# Autodesk Inventor assembly: Assembly.
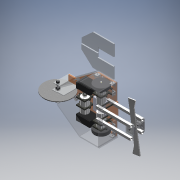
[picture p0: Inventor's stored thumbnail of the model, 180x180]
Saved by Autodesk Inventor 2019 (Build 230136000, 136)
## iProperties
Created: 2018-08-16
Part Number: Assembly.
Document SubType Name: Assembly
Designer: andres2416
Author: andres2416
## Documents named in this file (26)
- C:\Users\garstka1245\Downloads\bot\full-bot-assembly.iam
- C:\Users\garstka1245\Downloads\bot\Electronics\battery.ipt
- C:\Users\garstka1245\Downloads\bot\Motor Mount H\motor-mount-h-E30-bot.ipt
- C:\Users\garstka1245\Downloads\bot\Motor Mount H\motor-mount-h-E30-top.ipt
- C:\Users\garstka1245\Downloads\bot\Mechanicals\motor-E30-400.ipt
- C:\Users\garstka1245\Downloads\bot\Structure\bar-aluminium.ipt
- C:\Users\garstka1245\Downloads\bot\Structure\standoff.ipt
- C:\Users\garstka1245\Downloads\bot\Weapon Saw\wall-side-saw.ipt
- C:\Users\garstka1245\Downloads\bot\Weapon Saw\wall-saw-support.ipt
- C:\Users\garstka1245\Downloads\bot\Weapon Saw\wall-side-saw-hole.ipt
- C:\Users\garstka1245\Downloads\bot\Weapon Saw\weapon-saw.ipt
- C:\Users\garstka1245\Downloads\bot\Mechanicals\wheel-6in.ipt
- C:\Users\garstka1245\Downloads\bot\Weapon Saw\axle-saw.ipt
- C:\Users\garstka1245\Downloads\bot\Shell\base\base.ipt
- C:\Users\garstka1245\Downloads\bot\Shell\second-layer\platform.ipt
- C:\Users\garstka1245\Downloads\bot\Mechanicals\gear-vex.ipt
- C:\Users\garstka1245\Downloads\bot\Weapon Saw\axle-shaft-collar-saw.ipt
- C:\Users\garstka1245\Downloads\bot\Weapon Spinner\mount-point.ipt
- C:\Users\garstka1245\Downloads\bot\Weapon Spinner\axle-spinner.ipt
- C:\Users\garstka1245\Downloads\bot\Weapon Spinner\weapon-spinner.ipt
- C:\Users\garstka1245\Downloads\bot\Shell\wall-parts\wall-spinner.ipt
- C:\Users\garstka1245\Downloads\bot\Shell\wall-parts\wall-side.ipt
- C:\Users\garstka1245\Downloads\bot\Shell\wall-parts\wall-angled.ipt
- C:\Users\garstka1245\Downloads\bot\Structure\bracket-aluminium.ipt
- C:\Users\garstka1245\Downloads\bot\Motor Mount V\motor-mount-v-E30.ipt
- C:\Users\garstka1245\Downloads\bot\Mechanicals\pillowblock.ipt
## Components (61 placed, 25 different names)
1. battery:1 — Mate:116
2. battery:3 — Mate:115
3. wheel-6in:2 — Mate:89, Mate:124
4. wheel-6in:1 — Mate:105, Mate:125
5. gear-vex:1 — Mate:58, Flush:14, Rotation:1, Rotation:2, Rotation:4, Mate:126
6. gear-vex:2 — Mate:92, Flush:14, Rotation:1, Flush:15
7. pillowblock:1 — Mate:112, Mate:113
8. pillowblock:2 — Mate:110, Mate:111, Angle:1
9. motor-E30-400:1 — Mate:101, Mate:102, Mate:105, Flush:18, Mate:125
10. motor-E30-400:2 — Mate:87, Mate:88, Mate:89, Flush:17, Mate:124
11. motor-E30-400:3 — Mate:21, Mate:23, Mate:92, Flush:15, Flush:16
12. motor-mount-h-E30-bot:1 — Mate:96, Mate:97, Mate:98, Mate:99, Mate:102, Mate:107
13. motor-mount-h-E30-bot:2 — Mate:93, Mate:94, Mate:95, Mate:100, Mate:101, Mate:106, Flush:18
14. motor-mount-h-E30-top:2 — Mate:79, Mate:80, Mate:81
15. motor-mount-h-E30-bot:3 — Mate:79, Mate:80, Mate:81, Mate:86, Mate:88, Mate:104
16. motor-mount-h-E30-top:3 — Mate:82, Mate:83, Mate:84
17. motor-mount-h-E30-bot:4 — Mate:82, Mate:83, Mate:84, Mate:85, Mate:87, Mate:103, Flush:17
18. motor-mount-h-E30-bot:5 — Mate:23, Mate:24, Mate:25, Mate:27, Mate:91, Mate:122
19. motor-mount-h-E30-top:7 — Mate:25, Mate:27, Mate:122, Flush:16
20. motor-mount-h-E30-bot:6 — Mate:21, Mate:22, Mate:26, Mate:28, Mate:90, Mate:121
21. motor-mount-h-E30-top:8 — Mate:26, Mate:28, Mate:121
22. motor-mount-h-E30-top:5 — Mate:96, Mate:97, Mate:98
23. motor-mount-h-E30-top:6 — Mate:93, Mate:94, Mate:95
24. motor-mount-v-E30:1 — Mate:118
25. platform:2 — Angle:3, Mate:119
26. platform:1 — Angle:2, Mate:120
27. base:1 — Mate:1, Mate:2, Mate:3, Mate:4, Mate:5, Mate:6, Mate:7, Mate:8, Mate:9, Mate:10, Mate:11, Mate:12, Mate:13, Mate:14, Mate:15, Mate:16, Mate:17, Mate:18, Mate:19, Mate:22, Mate:24, Mate:46, Mate:47, Mate:48, Mate:51, Mate:52, Mate:53, Mate:62, Mate:65, Mate:66, Mate:67, Flush:4, Flush:5, Mate:71, Mate:73, Mate:76, Mate:85, Mate:86, Mate:90, Mate:91, Mate:99, Mate:100, Mate:103, Mate:104, Mate:106, Mate:107, Flush:10, Mate:108, Flush:11, Flush:13, Mate:109, Mate:115, Mate:116, Mate:118, Mate:119, Mate:120
28. wall-side:1 — Mate:73, Mate:74, Mate:75, Angle:3
29. wall-side:2 — Mate:60, Mate:61, Mate:62, Angle:2
30. wall-spinner:1 — Mate:76, Mate:77, Mate:78
31. wall-angled:2 — Mate:70, Mate:71, Mate:72
32. wall-angled:1 — Mate:63, Mate:64, Mate:65
33. standoff:4 — Mate:29, Mate:35, Mate:38, Mate:39
34. standoff:3 — Mate:31, Mate:33
35. standoff:2 — Mate:36, Mate:43
36. standoff:1 — Mate:37, Mate:40, Mate:41, Mate:42
37. bar-aluminium:1 — Mate:33, Mate:35, Mate:38, Flush:6, Flush:7, Mate:68
38. bar-aluminium:2 — Mate:36, Mate:37, Mate:40, Mate:51, Mate:52, Mate:53, Mate:114
39. bar-aluminium:3 — Mate:29, Mate:31, Mate:39, Mate:46, Mate:47, Mate:48, Flush:8, Flush:9
40. bar-aluminium:4 — Mate:41, Mate:42, Mate:43
41. bracket-aluminium:1 — Mate:15, Mate:64, Mate:66
42. bracket-aluminium:2 — Mate:12, Mate:16, Mate:63
43. bracket-aluminium:3 — Mate:11, Mate:14, Mate:72
44. bracket-aluminium:4 — Mate:6, Mate:8, Mate:70
45. bracket-aluminium:5 — Mate:9, Mate:19, Mate:78
46. bracket-aluminium:6 — Mate:1, Mate:2, Mate:77
47. bracket-aluminium:7 — Mate:10, Mate:18, Mate:61
48. bracket-aluminium:8 — Mate:13, Mate:17, Mate:60
49. bracket-aluminium:9 — Mate:3, Mate:4, Mate:74
50. bracket-aluminium:10 — Mate:5, Mate:7, Mate:75
51. wall-side-saw-hole:1 — Mate:55, Flush:10, Mate:108, Flush:11, Flush:12, Mate:126, Mate:127, Mate:128
52. wall-saw-support:1 — Mate:59, Flush:13, Mate:109, Mate:123
53. wall-side-saw:1 — Mate:67, Flush:4, Flush:5
54. weapon-saw:1 — Mate:54, Rotation:3, Mate:123
55. axle-saw:1 — Mate:54, Mate:55, Mate:56, Mate:57, Mate:58, Mate:59, Flush:12, Rotation:2, Rotation:3
56. axle-shaft-collar-saw:1 — Mate:56, Rotation:4, Rotation:5, Mate:127
57. axle-shaft-collar-saw:2 — Mate:57, Rotation:5, Mate:128
58. mount-point:1 — Flush:2, Mate:44, Flush:6, Flush:7, Mate:68, Mate:111, Angle:1
59. mount-point:2 — Mate:45, Flush:8, Flush:9, Mate:113, Mate:114
60. axle-spinner:1 — Mate:20, Flush:1, Flush:2, Mate:44, Mate:45, Mate:110, Mate:112
61. weapon-spinner:1 — Mate:20, Flush:1
## Relationships (146: Mate 121, Flush 17, RelateRotation 5, Angle 3)
- Mate:1: base:1 ↔ bracket-aluminium:6
- Mate:2: base:1 ↔ bracket-aluminium:6
- Mate:3: base:1 ↔ bracket-aluminium:9
- Mate:4: base:1 ↔ bracket-aluminium:9
- Mate:5: base:1 ↔ bracket-aluminium:10
- Mate:6: base:1 ↔ bracket-aluminium:4
- Mate:7: base:1 ↔ bracket-aluminium:10
- Mate:8: base:1 ↔ bracket-aluminium:4
- Mate:9: base:1 ↔ bracket-aluminium:5
- Mate:10: base:1 ↔ bracket-aluminium:7
- Mate:11: base:1 ↔ bracket-aluminium:3
- Mate:12: base:1 ↔ bracket-aluminium:2
- Mate:13: base:1 ↔ bracket-aluminium:8
- Mate:14: base:1 ↔ bracket-aluminium:3
- Mate:15: base:1 ↔ bracket-aluminium:1
- Mate:16: base:1 ↔ bracket-aluminium:2
- Mate:17: base:1 ↔ bracket-aluminium:8
- Mate:18: base:1 ↔ bracket-aluminium:7
- Mate:19: base:1 ↔ bracket-aluminium:5
- Mate:20: axle-spinner:1 ↔ weapon-spinner:1
- Flush:1 (50.8 mm): axle-spinner:1 ↔ weapon-spinner:1
- Mate:21: motor-E30-400:3 ↔ motor-mount-h-E30-bot:6
- Mate:22: motor-mount-h-E30-bot:6 ↔ base:1
- Mate:23: motor-E30-400:3 ↔ motor-mount-h-E30-bot:5
- Mate:24: motor-mount-h-E30-bot:5 ↔ base:1
- Mate:25: motor-mount-h-E30-bot:5 ↔ motor-mount-h-E30-top:7
- Mate:26: motor-mount-h-E30-bot:6 ↔ motor-mount-h-E30-top:8
- Mate:27: motor-mount-h-E30-bot:5 ↔ motor-mount-h-E30-top:7
- Mate:28: motor-mount-h-E30-bot:6 ↔ motor-mount-h-E30-top:8
- Mate:29: standoff:4 ↔ bar-aluminium:3
- Mate:31: standoff:3 ↔ bar-aluminium:3
- Mate:33: standoff:3 ↔ bar-aluminium:1
- Mate:35: standoff:4 ↔ bar-aluminium:1
- Mate:36: standoff:2 ↔ bar-aluminium:2
- Mate:37: standoff:1 ↔ bar-aluminium:2
- Mate:38: standoff:4 ↔ bar-aluminium:1
- Mate:39: standoff:4 ↔ bar-aluminium:3
- Mate:40: standoff:1 ↔ bar-aluminium:2
- Mate:41: standoff:1 ↔ bar-aluminium:4
- Mate:42: standoff:1 ↔ bar-aluminium:4
- Mate:43: standoff:2 ↔ bar-aluminium:4
- Flush:2: mount-point:1 ↔ axle-spinner:1
- Mate:44: mount-point:1 ↔ axle-spinner:1
- Mate:45: mount-point:2 ↔ axle-spinner:1
- Mate:46: base:1 ↔ bar-aluminium:3
- Mate:47: base:1 ↔ bar-aluminium:3
- Mate:48: base:1 ↔ bar-aluminium:3
- Mate:51: base:1 ↔ bar-aluminium:2
- Mate:52: base:1 ↔ bar-aluminium:2
- Mate:53: base:1 ↔ bar-aluminium:2
- Mate:54: weapon-saw:1 ↔ axle-saw:1
- Mate:55: wall-side-saw-hole:1 ↔ axle-saw:1
- Mate:56: axle-saw:1 ↔ axle-shaft-collar-saw:1
- Mate:57: axle-saw:1 ↔ axle-shaft-collar-saw:2
- Mate:58: gear-vex:1 ↔ axle-saw:1
- Mate:59: wall-saw-support:1 ↔ axle-saw:1
- Mate:60: wall-side:2 ↔ bracket-aluminium:8
- Mate:61: wall-side:2 ↔ bracket-aluminium:7
- Mate:62: base:1 ↔ wall-side:2
- Mate:63: wall-angled:1 ↔ bracket-aluminium:2
- Mate:64: wall-angled:1 ↔ bracket-aluminium:1
- Mate:65: base:1 ↔ wall-angled:1
- Mate:66: base:1 ↔ bracket-aluminium:1
- Mate:67: base:1 ↔ wall-side-saw:1
- Flush:4: base:1 ↔ wall-side-saw:1
- Flush:5: base:1 ↔ wall-side-saw:1
- Flush:6: bar-aluminium:1 ↔ mount-point:1
- Flush:7 (12.7 mm): bar-aluminium:1 ↔ mount-point:1
- Mate:68: bar-aluminium:1 ↔ mount-point:1
- Flush:8: bar-aluminium:3 ↔ mount-point:2
- Flush:9 (12.7 mm): bar-aluminium:3 ↔ mount-point:2
- Mate:70: wall-angled:2 ↔ bracket-aluminium:4
- Mate:71: base:1 ↔ wall-angled:2
- Mate:72: wall-angled:2 ↔ bracket-aluminium:3
- Mate:73: base:1 ↔ wall-side:1
- Mate:74: wall-side:1 ↔ bracket-aluminium:9
- Mate:75: wall-side:1 ↔ bracket-aluminium:10
- Mate:76: base:1 ↔ wall-spinner:1
- Mate:77: wall-spinner:1 ↔ bracket-aluminium:6
- Mate:78: wall-spinner:1 ↔ bracket-aluminium:5
- Mate:79: motor-mount-h-E30-top:2 ↔ motor-mount-h-E30-bot:3
- Mate:80: motor-mount-h-E30-top:2 ↔ motor-mount-h-E30-bot:3
- Mate:81: motor-mount-h-E30-top:2 ↔ motor-mount-h-E30-bot:3
- Mate:82: motor-mount-h-E30-top:3 ↔ motor-mount-h-E30-bot:4
- Mate:83: motor-mount-h-E30-top:3 ↔ motor-mount-h-E30-bot:4
- Mate:84: motor-mount-h-E30-top:3 ↔ motor-mount-h-E30-bot:4
- Mate:85: motor-mount-h-E30-bot:4 ↔ base:1
- Mate:86: motor-mount-h-E30-bot:3 ↔ base:1
- Mate:87: motor-E30-400:2 ↔ motor-mount-h-E30-bot:4
- Mate:88: motor-E30-400:2 ↔ motor-mount-h-E30-bot:3
- Mate:89: wheel-6in:2 ↔ motor-E30-400:2
- Mate:90: motor-mount-h-E30-bot:6 ↔ base:1
- Mate:91: motor-mount-h-E30-bot:5 ↔ base:1
- Mate:92: gear-vex:2 ↔ motor-E30-400:3
- Mate:93: motor-mount-h-E30-bot:2 ↔ motor-mount-h-E30-top:6
- Mate:94: motor-mount-h-E30-bot:2 ↔ motor-mount-h-E30-top:6
- Mate:95: motor-mount-h-E30-bot:2 ↔ motor-mount-h-E30-top:6
- Mate:96: motor-mount-h-E30-bot:1 ↔ motor-mount-h-E30-top:5
- Mate:97: motor-mount-h-E30-bot:1 ↔ motor-mount-h-E30-top:5
- Mate:98: motor-mount-h-E30-bot:1 ↔ motor-mount-h-E30-top:5
- Mate:99: motor-mount-h-E30-bot:1 ↔ base:1
- Mate:100: motor-mount-h-E30-bot:2 ↔ base:1
- Mate:101: motor-E30-400:1 ↔ motor-mount-h-E30-bot:2
- Mate:102: motor-E30-400:1 ↔ motor-mount-h-E30-bot:1
- Mate:103: motor-mount-h-E30-bot:4 ↔ base:1
- Mate:104: motor-mount-h-E30-bot:3 ↔ base:1
- Mate:105: wheel-6in:1 ↔ motor-E30-400:1
- Mate:106: motor-mount-h-E30-bot:2 ↔ base:1
- Mate:107: motor-mount-h-E30-bot:1 ↔ base:1
- Flush:10: base:1 ↔ wall-side-saw-hole:1
- Mate:108: base:1 ↔ wall-side-saw-hole:1
- Flush:11: base:1 ↔ wall-side-saw-hole:1
- Flush:12 (-25.4 mm): wall-side-saw-hole:1 ↔ axle-saw:1
- Flush:13: base:1 ↔ wall-saw-support:1
- Mate:109: base:1 ↔ wall-saw-support:1
- Mate:110: pillowblock:2 ↔ axle-spinner:1
- Mate:111: pillowblock:2 ↔ mount-point:1
- Angle:1 (0 deg): pillowblock:2 ↔ mount-point:1
- Mate:112: pillowblock:1 ↔ axle-spinner:1
- Mate:113: pillowblock:1 ↔ mount-point:2
- Mate:114: bar-aluminium:2 ↔ mount-point:2
- Mate:115: battery:3 ↔ base:1
- Mate:116: battery:1 ↔ base:1
- Flush:14: gear-vex:1 ↔ gear-vex:2
- Rotation:1 [RelateRotation] (1 ul): gear-vex:1 ↔ gear-vex:2
- Rotation:2 [RelateRotation] (1.6 ul): gear-vex:1 ↔ axle-saw:1
- Rotation:3 [RelateRotation] (19.2 ul): weapon-saw:1 ↔ axle-saw:1
- Mate:118: motor-mount-v-E30:1 ↔ base:1
- Angle:2 (0 deg): platform:1 ↔ wall-side:2
- Angle:3 (0 deg): platform:2 ↔ wall-side:1
- Mate:119: platform:2 ↔ base:1
- Mate:120: platform:1 ↔ base:1
- Flush:15: gear-vex:2 ↔ motor-E30-400:3
- Rotation:4 [RelateRotation] (1 ul): gear-vex:1 ↔ axle-shaft-collar-saw:1
- Rotation:5 [RelateRotation] (1 ul): axle-shaft-collar-saw:1 ↔ axle-shaft-collar-saw:2
- Mate:121: motor-mount-h-E30-bot:6 ↔ motor-mount-h-E30-top:8
- Mate:122: motor-mount-h-E30-bot:5 ↔ motor-mount-h-E30-top:7
- Flush:16: motor-E30-400:3 ↔ motor-mount-h-E30-top:7
- Mate:123: wall-saw-support:1 ↔ weapon-saw:1
- Flush:17: motor-E30-400:2 ↔ motor-mount-h-E30-bot:4
- Mate:124: wheel-6in:2 ↔ motor-E30-400:2
- Flush:18: motor-E30-400:1 ↔ motor-mount-h-E30-bot:2
- Mate:125: wheel-6in:1 ↔ motor-E30-400:1
- Mate:126: gear-vex:1 ↔ wall-side-saw-hole:1
- Mate:127: wall-side-saw-hole:1 ↔ axle-shaft-collar-saw:1
- Mate:128: wall-side-saw-hole:1 ↔ axle-shaft-collar-saw:2
